# Autodesk Inventor assembly: Skirts
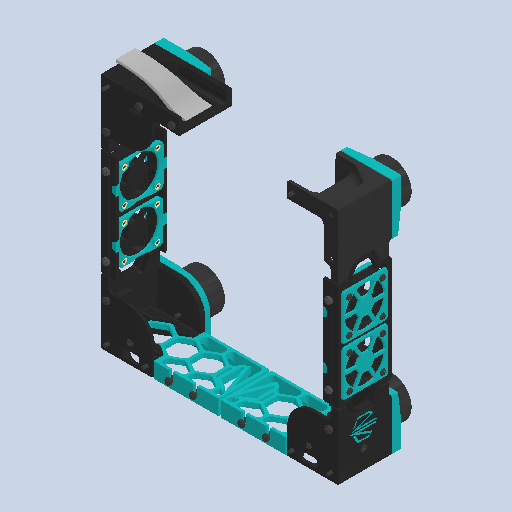
[picture p0: Inventor's stored thumbnail of the model, 512x512]
Saved by Autodesk Inventor 2026 (Build 300175050, 175E)
## iProperties
Created: 2025-07-29
Part Number: Skirts
Document SubType Name: Assembly
Designer: tdxt
Author: tdxt
## Documents named in this file (13)
- D:\Github\Pandoras_Box\CAD\pandoras_box_R2\pandoras_box_R2\Skirts.iam
- D:\Github\Pandoras_Box\CAD\pandoras_box_R2\pandoras_box_R2\leg_front_right v14.iam
- D:\Github\Pandoras_Box\CAD\pandoras_box_R2\pandoras_box_R2\leg_rear v10.iam
- D:\Github\Pandoras_Box\CAD\pandoras_box_R2\pandoras_box_R2\Leg - Front Left.iam
- D:\Github\Pandoras_Box\CAD\pandoras_box_R2\pandoras_box_R2\Side Skirt v4.iam
- D:\Github\Pandoras_Box\CAD\pandoras_box_R2\pandoras_box_R2\Front Skirt v23.iam
- D:\Github\Pandoras_Box\CAD\pandoras_box_R2\pandoras_box_R2\Skirt_Front_Mirror.iam
- D:\Github\Pandoras_Box\CAD\pandoras_box_R2\pandoras_box_R2\Corner_A v11.iam
- D:\Github\Pandoras_Box\CAD\pandoras_box_R2\pandoras_box_R2\Foot v8(Mirror).iam
- D:\Github\Pandoras_Box\CAD\pandoras_box_R2\pandoras_box_R2\Foot v8(Mirror)_1.iam
- D:\Github\Pandoras_Box\CAD\pandoras_box_R2\pandoras_box_R2\leg_mains_inlet v6.iam
- D:\Github\Pandoras_Box\CAD\pandoras_box_R2\pandoras_box_R2\Corner_A v11_1.iam
- D:\Github\Pandoras_Box\CAD\pandoras_box_R2\pandoras_box_R2\Side Skirt - Fan v4.iam
## Components (13 placed, 10 different names)
1. leg_front_right v14:1 [sub-assembly]
2. leg_rear v10:1 [sub-assembly] — 表面齐平:2
3. Leg - Front Left:1 [sub-assembly]
4. Side Skirt v4:1 [sub-assembly]
5. Front Skirt v23:1 [sub-assembly]
6. Skirt_Front_Mirror:1 [sub-assembly]
7. Corner_A v11:1 [sub-assembly]
8. Foot v8(Mirror):1 [sub-assembly]
9. Foot v8(Mirror):2 [sub-assembly]
10. leg_mains_inlet v6:1 [sub-assembly]
11. Corner_A v11:2 [sub-assembly]
12. Side Skirt - Fan v4:1 [sub-assembly] — 表面齐平:3, 表面齐平:4
13. Side Skirt - Fan v4:2 [sub-assembly] — 表面齐平:2, 表面齐平:3, 表面齐平:4
## Relationships (3: Flush 3)
- 表面齐平:2 [Flush]: leg_rear v10:1 ↔ Side Skirt - Fan v4:2
- 表面齐平:3 [Flush]: Side Skirt - Fan v4:1 ↔ Side Skirt - Fan v4:2
- 表面齐平:4 [Flush]: Side Skirt - Fan v4:1 ↔ Side Skirt - Fan v4:2
